# Autodesk Inventor assembly: basketwheel
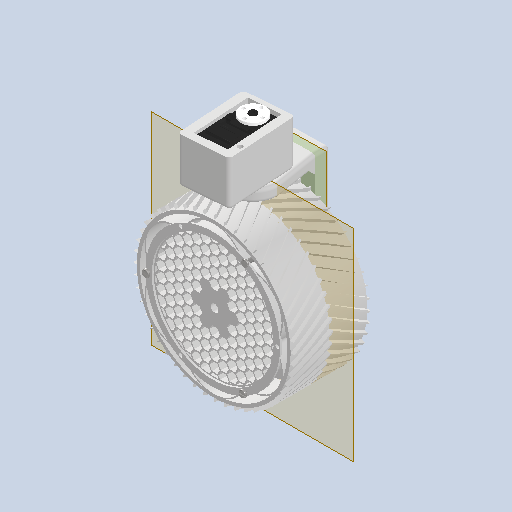
[picture p0: Inventor's stored thumbnail of the model, 512x512]
Saved by Autodesk Inventor 2025.3 (Build 293356000, 356)
## iProperties
Created: 2026-04-05
Part Number: basketwheel
Document SubType Name: Assembly
Designer: ksawe
Author: ksawe
## Documents named in this file (3)
- C:\Users\ksawe\OneDrive\Pulpit\Exomy v1\wersja2\basketwheel.iam
- C:\Users\ksawe\OneDrive\Pulpit\Exomy v1\wersja2\kolowahacz.iam
- C:\Users\ksawe\OneDrive\Pulpit\Exomy v1\wersja2\basketserwo.iam
## Components (2 placed, 2 different names)
1. kolowahacz:1 [sub-assembly] — Rotation:1, Insert:1
2. basketserwo:1 [sub-assembly] — Rotation:1, Insert:1
## Relationships (2: RelateRotation 1, Insert 1)
- Rotation:1 [RelateRotation] (0.64 ul): kolowahacz:1 ↔ basketserwo:1
- Insert:1: kolowahacz:1 ↔ basketserwo:1
